# Autodesk Inventor assembly: 32ch_ECoG_assembled
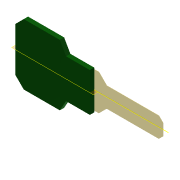
[picture p0: Inventor's stored thumbnail of the model, 180x180]
Saved by Autodesk Inventor 2014 (Build 180170000, 170)
## iProperties
Created: 2016-08-28
Part Number: 32ch_ECoG_assembled
Document SubType Name: Assembly
Designer: Camilo
Author: Camilo
## Documents named in this file (3)
- Z:\Github\AgingTests\3D parts\ECoG holder_2p0\32ch_ECoG_assembled.iam
- Z:\Github\AgingTests\3D parts\ECoG holder_2p0\32ch_ACF2TDT_board.ipt
- Z:\Github\AgingTests\3D parts\ECoG holder_2p0\32ch_ECoG.ipt
## Components (2 placed, 2 different names)
1. 32ch_ACF2TDT_board:1 — Mate:1, Flush:1, Flush:2, Mate:2, Mate:3, Mate:4
2. 32ch_ECoG:1 — Mate:2, Mate:3, Mate:4
## Relationships (6: Mate 4, Flush 2)
- Mate:1: 32ch_ACF2TDT_board:1
- Flush:1: 32ch_ACF2TDT_board:1
- Flush:2: 32ch_ACF2TDT_board:1
- Mate:2: 32ch_ACF2TDT_board:1 ↔ 32ch_ECoG:1
- Mate:3: 32ch_ACF2TDT_board:1 ↔ 32ch_ECoG:1
- Mate:4 (-6 mm): 32ch_ACF2TDT_board:1 ↔ 32ch_ECoG:1
